# Autodesk Inventor assembly: Mousetrap_Assembly_draft
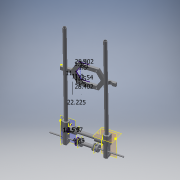
[picture p0: Inventor's stored thumbnail of the model, 180x180]
Saved by Autodesk Inventor 2018 (Build 220112000, 112)
## iProperties
Created: 2018-11-05
Part Number: Mousetrap_Assembly_draft
Document SubType Name: Assembly
Designer: Payal Jindal
Author: Payal Jindal
## Documents named in this file (9)
- C:\Users\Payal Jindal\Documents\Mousetrap18-19\Mousetrap_Assembly_draft.iam
- C:\Users\Payal Jindal\Documents\Mousetrap18-19\axle.ipt
- C:\Users\Payal Jindal\Documents\Mousetrap18-19\chassiswithdowel.ipt
- C:\Users\Payal Jindal\Documents\Mousetrap18-19\front_right_chassis.ipt
- C:\Users\Payal Jindal\Documents\Mousetrap18-19\long_carbon_fiber.ipt
- C:\Users\Payal Jindal\Documents\Mousetrap18-19\short_carbon_fiber.ipt
- C:\Users\Payal Jindal\Documents\Mousetrap18-19\spindles.ipt
- C:\Users\Payal Jindal\Documents\Mousetrap18-19\flange_bearing.ipt
- C:\Users\Payal Jindal\Documents\Inventor\Mousetrap2.0\Mousetrap holders.ipt
## Components (10 placed, 8 different names)
1. axle:1 — Mate:15, Mate:16
2. chassiswithdowel:1 — Mate:3, Mate:4, Mate:5, Mate:6, Mate:7, Mate:9, Mate:11, Mate:12, Mate:15
3. front_right_chassis:1 — Mate:1, Mate:2, Mate:5, Mate:6, Mate:8, Mate:10, Mate:13, Mate:14
4. long_carbon_fiber:1 — Mate:1, Mate:2
5. short_carbon_fiber:1 — Mate:7, Mate:8, Mate:9, Mate:10
6. spindles:1 — Mate:16
7. flange_bearing:1 — Mate:11, Mate:12
8. flange_bearing:2 — Mate:13, Mate:14
9. long_carbon_fiber:2 — Mate:3, Mate:4, Mate:17
10. Mousetrap holders:1 — Mate:17
## Relationships (17: Mate 17)
- Mate:1: front_right_chassis:1 ↔ long_carbon_fiber:1
- Mate:2: front_right_chassis:1 ↔ long_carbon_fiber:1
- Mate:3: chassiswithdowel:1 ↔ long_carbon_fiber:2
- Mate:4: chassiswithdowel:1 ↔ long_carbon_fiber:2
- Mate:5: chassiswithdowel:1 ↔ front_right_chassis:1
- Mate:6: chassiswithdowel:1 ↔ front_right_chassis:1
- Mate:7: chassiswithdowel:1 ↔ short_carbon_fiber:1
- Mate:8: front_right_chassis:1 ↔ short_carbon_fiber:1
- Mate:9: chassiswithdowel:1 ↔ short_carbon_fiber:1
- Mate:10: front_right_chassis:1 ↔ short_carbon_fiber:1
- Mate:11: chassiswithdowel:1 ↔ flange_bearing:1
- Mate:12: chassiswithdowel:1 ↔ flange_bearing:1
- Mate:13: front_right_chassis:1 ↔ flange_bearing:2
- Mate:14: front_right_chassis:1 ↔ flange_bearing:2
- Mate:15: axle:1 ↔ chassiswithdowel:1
- Mate:16: axle:1 ↔ spindles:1
- Mate:17: long_carbon_fiber:2 ↔ Mousetrap holders:1
